# Autodesk Inventor assembly: １段目アーム
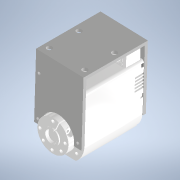
[picture p0: Inventor's stored thumbnail of the model, 180x180]
Saved by Autodesk Inventor 2022 (Build 260153000, 153)
## iProperties
Created: 2022-11-23
Part Number: １段目アーム
Document SubType Name: Assembly
Designer: tdn82
Author: tdn82
## Documents named in this file (3)
- C:\Users\tdn82\OneDrive\ドキュメント\Inventor\卒業研究パネル型スカラアーム\１段目アーム.iam
- C:\Users\tdn82\OneDrive\ドキュメント\Inventor\卒業研究パネル型スカラアーム\B3M1100_scale_step\サーボモータB3M-SC-1170-AB3M1100_scale.ipt
- C:\Users\tdn82\OneDrive\ドキュメント\Inventor\卒業研究パネル型スカラアーム\サーボモータ固定用.ipt
## Components (2 placed, 2 different names)
1. サーボモータ固定用:1 — 挿入:1, 挿入:2
2. サーボモータB3M-SC-1170-AB3M1100_scale:1 — 挿入:1, 挿入:2
## Relationships (2: Insert 2)
- 挿入:1 [Insert]: サーボモータ固定用:1 ↔ サーボモータB3M-SC-1170-AB3M1100_scale:1
- 挿入:2 [Insert]: サーボモータ固定用:1 ↔ サーボモータB3M-SC-1170-AB3M1100_scale:1
